# Autodesk Inventor assembly: candynamix_mini
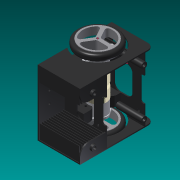
[picture p0: Inventor's stored thumbnail of the model, 180x180]
Saved by Autodesk Inventor 2015 (Build 190159000, 159)
## iProperties
Created: 2018-12-01
Part Number: candynamix_mini
Document SubType Name: Assembly
Designer: tlsru
Author: tlsru
## Documents named in this file (7)
- D:\00_[sigma project]\CanRobot_Project\01_[CAD] Inventor\2018_candynamix_mini\candynamix_mini.iam
- D:\00_[sigma project]\CanRobot_Project\01_[CAD] Inventor\2018_candynamix_mini\GM15BY_StepperMotor.ipt
- D:\00_[sigma project]\CanRobot_Project\01_[CAD] Inventor\2018_candynamix_mini\n2_miniWheel.ipt
- D:\00_[sigma project]\CanRobot_Project\01_[CAD] Inventor\2018_candynamix_mini\BATTARY HOLDER.ipt
- D:\00_[sigma project]\CanRobot_Project\01_[CAD] Inventor\2018_candynamix_mini\candynamix_mini_base.ipt
- D:\00_[sigma project]\CanRobot_Project\01_[CAD] Inventor\2018_candynamix_mini\Orangepi\Imported Components\Orange Pi Zero v1_1 - Ensamblaje\Orange Pi Zero v1_1 - Ensamblaje.iam
- D:\00_[sigma project]\CanRobot_Project\01_[CAD] Inventor\2018_candynamix_mini\candynamix_mini_ballcaster.ipt
## Components (8 placed, 6 different names)
1. GM15BY_StepperMotor:1 — 삽입:1, 삽입:3
2. n2_miniWheel:1 — 삽입:1
3. GM15BY_StepperMotor:2 — 삽입:2, 삽입:4
4. n2_miniWheel:2 — 삽입:2
5. BATTARY HOLDER:1 — 메이트:1, 메이트:2, 메이트:3
6. candynamix_mini_base:1 — 메이트:1, 메이트:2, 메이트:3, 메이트:4, 플러쉬:2, 플러쉬:3, 플러쉬:4, 삽입:3, 삽입:4
7. Orange Pi Zero v1_1 - Ensamblaje:1 [sub-assembly] — 메이트:4, 플러쉬:2, 플러쉬:3
8. candynamix_mini_ballcaster:1 — 플러쉬:4
## Relationships (11: Insert 4, Mate 4, Flush 3)
- 삽입:1 [Insert] (0.5 mm): GM15BY_StepperMotor:1 ↔ n2_miniWheel:1
- 삽입:2 [Insert] (0.5 mm): GM15BY_StepperMotor:2 ↔ n2_miniWheel:2
- 메이트:1 [Mate]: BATTARY HOLDER:1 ↔ candynamix_mini_base:1
- 메이트:2 [Mate] (2 mm): BATTARY HOLDER:1 ↔ candynamix_mini_base:1
- 메이트:3 [Mate] (1 mm): BATTARY HOLDER:1 ↔ candynamix_mini_base:1
- 메이트:4 [Mate] (3.5 mm): candynamix_mini_base:1 ↔ Orange Pi Zero v1_1 - Ensamblaje:1
- 플러쉬:2 [Flush] (-5 mm): candynamix_mini_base:1 ↔ Orange Pi Zero v1_1 - Ensamblaje:1
- 플러쉬:3 [Flush]: candynamix_mini_base:1 ↔ Orange Pi Zero v1_1 - Ensamblaje:1
- 플러쉬:4 [Flush]: candynamix_mini_base:1 ↔ candynamix_mini_ballcaster:1
- 삽입:3 [Insert]: GM15BY_StepperMotor:1 ↔ candynamix_mini_base:1
- 삽입:4 [Insert]: GM15BY_StepperMotor:2 ↔ candynamix_mini_base:1
